# Autodesk Inventor assembly: OBUDOWA TYLNA MONITORA + ZŁĄCZA
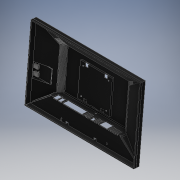
[picture p0: Inventor's stored thumbnail of the model, 180x180]
Saved by Autodesk Inventor 2017 SP1 (Build 210196100, 196)
## iProperties
Created: 2021-03-07
Part Number: OBUDOWA TYLNA MONITORA + ZŁĄCZA
Document SubType Name: Assembly
Designer: Administrator
Author: Administrator
## Documents named in this file (6)
- D:\PRYWATNE\PROJEKTY\POKÓJ\URZĄDZENIA PERYFERYJNE\DELL 1909Wf\OBUDOWA TYLNA MONITORA + ZŁĄCZA.iam
- D:\PRYWATNE\PROJEKTY\POKÓJ\URZĄDZENIA PERYFERYJNE\DELL 1909Wf\OBUDOWAN TYLNA MONITORA.ipt
- D:\PRYWATNE\PROJEKTY\POKÓJ\URZĄDZENIA PERYFERYJNE\DELL 1909Wf\ZŁĄCZA\USB A 2.0\femaleThruHoleUSB.ipt
- D:\PRYWATNE\PROJEKTY\POKÓJ\URZĄDZENIA PERYFERYJNE\DELL 1909Wf\WYSUWANY PLASTIK.ipt
- C:\Users\Administrator\Documents\Inventor\Content Center Files\R2017\pl-PL\DIN 7985 (H)\DIN 7985 (H) - M4x5-H.ipt
- D:\PRYWATNE\PROJEKTY\POKÓJ\URZĄDZENIA PERYFERYJNE\DELL 1909Wf\SPUST.ipt
## Components (9 placed, 5 different names)
1. OBUDOWAN TYLNA MONITORA:1 — Wstaw:1, Wstaw:2, Wstaw:3, Wstaw:4, Równoległy:2
2. femaleThruHoleUSB:1
3. femaleThruHoleUSB:2
4. WYSUWANY PLASTIK:1
5. DIN 7985 (H) M4x5-H:1 — Wstaw:1
6. DIN 7985 (H) M4x5-H:2 — Wstaw:2
7. DIN 7985 (H) M4x5-H:3 — Wstaw:3
8. DIN 7985 (H) M4x5-H:4 — Wstaw:4
9. SPUST:1 — Równoległy:2
## Relationships (10: Mate 4, Insert 4, Flush 2)
- [Mate] (0.75 mm): OBUDOWAN TYLNA MONITORA:1 ↔ femaleThruHoleUSB:1
- [Mate] (0.645 mm): OBUDOWAN TYLNA MONITORA:1 ↔ femaleThruHoleUSB:1
- [Mate] (0.75 mm): OBUDOWAN TYLNA MONITORA:1 ↔ femaleThruHoleUSB:2
- [Mate] (0.645 mm): OBUDOWAN TYLNA MONITORA:1 ↔ femaleThruHoleUSB:2
- [Flush]: OBUDOWAN TYLNA MONITORA:1 ↔ WYSUWANY PLASTIK:1
- Wstaw:1 [Insert]: OBUDOWAN TYLNA MONITORA:1 ↔ DIN 7985 (H) M4x5-H:1
- Wstaw:2 [Insert]: OBUDOWAN TYLNA MONITORA:1 ↔ DIN 7985 (H) M4x5-H:2
- Wstaw:3 [Insert]: OBUDOWAN TYLNA MONITORA:1 ↔ DIN 7985 (H) M4x5-H:3
- Wstaw:4 [Insert]: OBUDOWAN TYLNA MONITORA:1 ↔ DIN 7985 (H) M4x5-H:4
- Równoległy:2 [Flush]: OBUDOWAN TYLNA MONITORA:1 ↔ SPUST:1
